# Autodesk Inventor assembly: Assembly
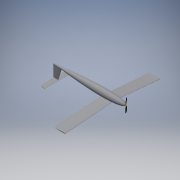
[picture p0: Inventor's stored thumbnail of the model, 180x180]
Saved by Autodesk Inventor 2019 (Build 230136000, 136)
## iProperties
Created: 2019-04-06
Part Number: Assembly
Document SubType Name: Assembly
Designer: albaa
Mass: 1699.02 g
Surface Area: 21119.3 cm^2
Volume: 7570.8 cm^3
Density: 0.224417 g/cm^3
Author: albaa
## Documents named in this file (9)
- C:\Users\albaa\Google Drive\McGill OneDrive\McGill\Courses\13_WINTER 2019\MECH 532\Project\REPO_mech532-project\CAD\Assembly.iam
- C:\Users\albaa\Google Drive\McGill OneDrive\McGill\Courses\13_WINTER 2019\MECH 532\Project\REPO_mech532-project\CAD\hTail_wing.ipt
- C:\Users\albaa\Google Drive\McGill OneDrive\McGill\Courses\13_WINTER 2019\MECH 532\Project\REPO_mech532-project\CAD\main_wing.ipt
- C:\Users\albaa\Google Drive\McGill OneDrive\McGill\Courses\13_WINTER 2019\MECH 532\Project\REPO_mech532-project\CAD\vTail_wing.ipt
- C:\Users\albaa\Google Drive\McGill OneDrive\McGill\Courses\13_WINTER 2019\MECH 532\Project\REPO_mech532-project\CAD\motor.ipt
- C:\Users\albaa\Google Drive\McGill OneDrive\McGill\Courses\13_WINTER 2019\MECH 532\Project\REPO_mech532-project\CAD\propeller.ipt
- C:\Users\albaa\Google Drive\McGill OneDrive\McGill\Courses\13_WINTER 2019\MECH 532\Project\REPO_mech532-project\CAD\battery.ipt
- C:\Users\albaa\Google Drive\McGill OneDrive\McGill\Courses\13_WINTER 2019\MECH 532\Project\REPO_mech532-project\CAD\payload.ipt
- C:\Users\albaa\Google Drive\McGill OneDrive\McGill\Courses\13_WINTER 2019\MECH 532\Project\REPO_mech532-project\CAD\fuselage_2.ipt
## Components (8 placed, 8 different names)
1. fuselage_2:1 — Mate:1, Mate:2, Flush:14, Flush:15, Mate:3, Flush:16, Flush:8, Flush:6, Tangent:1, Flush:17, Flush:18, Flush:19, Mate:8, Mate:9
2. hTail_wing:1 — Flush:6, Mate:2, Flush:15
3. main_wing:1 — Mate:1, Mate:3, Flush:16
4. vTail_wing:1 — Flush:8, Flush:14
5. motor:1 — Mate:5, Mate:6, Tangent:1
6. propeller:1 — Mate:5, Mate:6
7. battery:1 — Mate:7, Flush:17, Flush:19
8. payload:1 — Mate:7, Flush:18
## Relationships (23: Flush 13, Mate 9, Tangent 1)
- [Flush]: fuselage_2:1
- Mate:1 (-500 mm): fuselage_2:1 ↔ main_wing:1
- Flush:6 (-250 mm): fuselage_2:1 ↔ hTail_wing:1
- Mate:2 (-1400 mm): fuselage_2:1 ↔ hTail_wing:1
- [Flush]: fuselage_2:1 ↔ vTail_wing:1
- Flush:8: fuselage_2:1 ↔ vTail_wing:1
- [Flush]: fuselage_2:1
- Mate:3 (70 mm): fuselage_2:1 ↔ main_wing:1
- [Mate]: fuselage_2:1 ↔ motor:1
- Mate:5: motor:1 ↔ propeller:1
- Mate:6: motor:1 ↔ propeller:1
- [Flush]: fuselage_2:1 ↔ battery:1
- [Flush]: fuselage_2:1 ↔ payload:1
- Flush:14 (-1340 mm): fuselage_2:1 ↔ vTail_wing:1
- Flush:15: fuselage_2:1 ↔ hTail_wing:1
- Flush:16: fuselage_2:1 ↔ main_wing:1
- Tangent:1: fuselage_2:1 ↔ motor:1
- Mate:7: battery:1 ↔ payload:1
- Flush:17 (10 mm): fuselage_2:1 ↔ battery:1
- Flush:18 (-360 mm): fuselage_2:1 ↔ payload:1
- Flush:19 (325 mm): fuselage_2:1 ↔ battery:1
- Mate:8: fuselage_2:1
- Mate:9: fuselage_2:1
## Named parameters: hWing_hOffset = 1150 mm, vWing_hOffset = 1090 mm, mainWing_vOffset = 70 mm, hWing_vOffset = 250 mm, vWing_height = 250 mm, battery_hOffset = 325 mm, battery_vOffset = -10 mm, mainWing_hOffset = 500 mm, payload_hOffset = 360 mm
